# Autodesk Inventor assembly: MovingArm
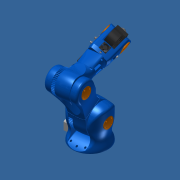
[picture p0: Inventor's stored thumbnail of the model, 180x180]
Saved by Autodesk Inventor 2014 SP2 (Build 180246200, 246)
## iProperties
Created: 2014-12-13
Part Number: MovingArm
Document SubType Name: Assembly
Designer: 4ndreas
Author: 4ndreas
## Documents named in this file (22)
- C:\Users\4ndreas\Documents\Inventor\RobotARm\MovingArm.iam
- C:\Users\4ndreas\Documents\Inventor\RobotARm\Nema17.ipt
- C:\Users\4ndreas\Documents\Inventor\Content Center Files\R2014\de-DE\DIN BEARING(1)\DIN 625 SKF - SKF 608.ipt
- C:\Users\4ndreas\Documents\Inventor\Content Center Files\R2014\de-DE\DIN 931-1\DIN 931-1 - M8 x 60.ipt
- C:\Users\4ndreas\Documents\Inventor\RobotARm\ArmSegment_klein_Gear.ipt
- C:\Users\4ndreas\Documents\Inventor\RobotARm\ArmSegment_klein.ipt
- C:\Users\4ndreas\Documents\Inventor\RobotARm\Nema17 Geared.ipt
- C:\Users\4ndreas\Documents\Inventor\RobotARm\Abdeckung.ipt
- C:\Users\4ndreas\Documents\Inventor\RobotARm\print\ArmPrint_A.ipt
- C:\Users\4ndreas\Documents\Inventor\RobotARm\print\ArmPrint_B_gear.ipt
- C:\Users\4ndreas\Documents\Inventor\RobotARm\print\ArmPrint_C_head.ipt
- C:\Users\4ndreas\Documents\Inventor\RobotARm\Stirnzahnrad_A_print.ipt
- C:\Users\4ndreas\Documents\Inventor\RobotARm\Stirnzahnrad_B_print.ipt
- C:\Users\4ndreas\Documents\Inventor\RobotARm\print\basis_print.ipt
- C:\Users\4ndreas\Documents\Inventor\RobotARm\foreArm.iam
- C:\Users\4ndreas\Documents\Inventor\Content Center Files\R2014\Leufter_30mm.ipt
- C:\Users\4ndreas\Documents\Inventor\RobotARm\MovingArm\AIP\FEA\b9sg0glls.fins
- C:\Users\4ndreas\Documents\Inventor\RobotARm\MovingArm\AIP\FEA\b9sg0glls.fsat
- C:\Users\4ndreas\Documents\Inventor\RobotARm\MovingArm\AIP\FEA\b9sg0glls.ftes
- C:\Users\4ndreas\Documents\Inventor\RobotARm\MovingArm\AIP\FEA\b9sg0glls.fwiz
- C:\Users\4ndreas\Documents\Inventor\RobotARm\MovingArm\AIP\FEA\b9sg0glxc.fmsh
- C:\Users\4ndreas\Documents\Inventor\RobotARm\MovingArm\AIP\FEA\b9sg0glxd.fres
## Components (23 placed, 15 different names)
1. basis_print:1 — Passend:1, Passend:2, Passend:4, Passend:6, Passend:7, Passend:8, Passend:9, Passend:10, Passend:11, Passend:12, Passend:13, Passend:14, Passend:43, Passend:44, Passend:45, Passend:46, Passend:47, Passend:48, Passend:50, Passend:69
2. Nema17:1 — Passend:5, Passend:6, Passend:67, Passend:69
3. DIN 625 SKF 608:1 — Passend:8, Passend:13
4. DIN 625 SKF 608:2 — Passend:7, Passend:14, Passend:15, Passend:18
5. DIN 625 SKF 608:3 — Passend:10, Passend:12, Passend:16, Passend:17
6. DIN 625 SKF 608:4 — Passend:9, Passend:11
7. DIN 931-1 - ersetzt durch DIN EN 24014 M8 x 60:1 — Passend:16, Passend:17, Passend:49
8. DIN 931-1 - ersetzt durch DIN EN 24014 M8 x 60:2 — Passend:15, Passend:18, Passend:51
9. Nema17:2 — Passend:56, Passend:59, Passend:60, Passend:68
10. ArmSegment_klein_Gear:1 — Passend:27, Passend:28, Passend:29, Passend:30, Passend:31, Passend:32, Passend:57, Passend:58, Fluchtend:3, Passend:72, Passend:73, Passend:76
11. ArmSegment_klein:1 — Passend:30, Passend:31, Passend:32, Passend:71
12. Nema17 Geared:1 — Passend:27, Passend:28, Passend:29, Passend:70
13. Abdeckung:1 — Passend:61, Passend:65, Passend:66
14. Abdeckung:2 — Passend:44, Passend:45, Passend:46
15. Abdeckung:3 — Passend:62, Passend:63, Passend:64
16. Abdeckung:4 — Passend:43, Passend:47, Passend:48
17. ArmPrint_A:1 — Passend:49, Passend:50, Passend:52, Fluchtend:1, Passend:55, Passend:62
18. ArmPrint_B_gear:1 — Passend:51, Passend:52, Fluchtend:1, Passend:53, Passend:54, Fluchtend:2
19. ArmPrint_C_head:1 — Passend:53, Passend:54, Passend:55, Passend:56, Passend:57, Passend:58, Passend:59, Passend:60, Passend:61, Passend:63, Passend:64, Passend:65, Passend:66
20. Stirnzahnrad_A_print:1 — Passend:67, Fluchtend:2
21. Stirnzahnrad_B_print:1 — Passend:68, Fluchtend:3
22. foreArm:1 [sub-assembly] — Passend:70, Passend:71
23. Leufter_30mm:1 — Passend:72, Passend:73, Passend:74, Passend:75
## Relationships (60: Mate 57, Flush 3)
- Passend:1 [Mate]: basis_print:1
- Passend:2 [Mate]: basis_print:1
- Passend:4 [Mate]: basis_print:1
- Passend:5 [Mate]: Nema17:1
- Passend:6 [Mate]: basis_print:1 ↔ Nema17:1
- Passend:7 [Mate]: basis_print:1 ↔ DIN 625 SKF 608:2
- Passend:8 [Mate]: basis_print:1 ↔ DIN 625 SKF 608:1
- Passend:9 [Mate]: basis_print:1 ↔ DIN 625 SKF 608:4
- Passend:10 [Mate]: basis_print:1 ↔ DIN 625 SKF 608:3
- Passend:11 [Mate]: basis_print:1 ↔ DIN 625 SKF 608:4
- Passend:12 [Mate]: basis_print:1 ↔ DIN 625 SKF 608:3
- Passend:13 [Mate]: basis_print:1 ↔ DIN 625 SKF 608:1
- Passend:14 [Mate]: basis_print:1 ↔ DIN 625 SKF 608:2
- Passend:15 [Mate]: DIN 625 SKF 608:2 ↔ DIN 931-1 - ersetzt durch DIN EN 24014 M8 x 60:2
- Passend:16 [Mate]: DIN 625 SKF 608:3 ↔ DIN 931-1 - ersetzt durch DIN EN 24014 M8 x 60:1
- Passend:17 [Mate]: DIN 625 SKF 608:3 ↔ DIN 931-1 - ersetzt durch DIN EN 24014 M8 x 60:1
- Passend:18 [Mate]: DIN 625 SKF 608:2 ↔ DIN 931-1 - ersetzt durch DIN EN 24014 M8 x 60:2
- Passend:27 [Mate]: ArmSegment_klein_Gear:1 ↔ Nema17 Geared:1
- Passend:28 [Mate]: ArmSegment_klein_Gear:1 ↔ Nema17 Geared:1
- Passend:29 [Mate]: ArmSegment_klein_Gear:1 ↔ Nema17 Geared:1
- Passend:30 [Mate]: ArmSegment_klein_Gear:1 ↔ ArmSegment_klein:1
- Passend:31 [Mate]: ArmSegment_klein_Gear:1 ↔ ArmSegment_klein:1
- Passend:32 [Mate]: ArmSegment_klein_Gear:1 ↔ ArmSegment_klein:1
- Passend:43 [Mate]: basis_print:1 ↔ Abdeckung:4
- Passend:44 [Mate]: basis_print:1 ↔ Abdeckung:2
- Passend:45 [Mate]: basis_print:1 ↔ Abdeckung:2
- Passend:46 [Mate]: basis_print:1 ↔ Abdeckung:2
- Passend:47 [Mate]: basis_print:1 ↔ Abdeckung:4
- Passend:48 [Mate]: basis_print:1 ↔ Abdeckung:4
- Passend:49 [Mate]: DIN 931-1 - ersetzt durch DIN EN 24014 M8 x 60:1 ↔ ArmPrint_A:1
- Passend:50 [Mate] (3 mm): basis_print:1 ↔ ArmPrint_A:1
- Passend:51 [Mate]: DIN 931-1 - ersetzt durch DIN EN 24014 M8 x 60:2 ↔ ArmPrint_B_gear:1
- Passend:52 [Mate]: ArmPrint_A:1 ↔ ArmPrint_B_gear:1
- Fluchtend:1 [Flush]: ArmPrint_A:1 ↔ ArmPrint_B_gear:1
- Passend:53 [Mate]: ArmPrint_B_gear:1 ↔ ArmPrint_C_head:1
- Passend:54 [Mate]: ArmPrint_B_gear:1 ↔ ArmPrint_C_head:1
- Passend:55 [Mate]: ArmPrint_A:1 ↔ ArmPrint_C_head:1
- Passend:56 [Mate]: Nema17:2 ↔ ArmPrint_C_head:1
- Passend:57 [Mate]: ArmSegment_klein_Gear:1 ↔ ArmPrint_C_head:1
- Passend:58 [Mate] (2 mm): ArmSegment_klein_Gear:1 ↔ ArmPrint_C_head:1
- Passend:59 [Mate]: Nema17:2 ↔ ArmPrint_C_head:1
- Passend:60 [Mate]: Nema17:2 ↔ ArmPrint_C_head:1
- Passend:61 [Mate]: Abdeckung:1 ↔ ArmPrint_C_head:1
- Passend:62 [Mate]: Abdeckung:3 ↔ ArmPrint_A:1
- Passend:63 [Mate]: Abdeckung:3 ↔ ArmPrint_C_head:1
- Passend:64 [Mate]: Abdeckung:3 ↔ ArmPrint_C_head:1
- Passend:65 [Mate]: Abdeckung:1 ↔ ArmPrint_C_head:1
- Passend:66 [Mate]: Abdeckung:1 ↔ ArmPrint_C_head:1
- Passend:67 [Mate]: Nema17:1 ↔ Stirnzahnrad_A_print:1
- Fluchtend:2 [Flush] (-1 mm): ArmPrint_B_gear:1 ↔ Stirnzahnrad_A_print:1
- Passend:68 [Mate]: Nema17:2 ↔ Stirnzahnrad_B_print:1
- Fluchtend:3 [Flush]: ArmSegment_klein_Gear:1 ↔ Stirnzahnrad_B_print:1
- Passend:69 [Mate]: basis_print:1 ↔ Nema17:1
- Passend:70 [Mate]: Nema17 Geared:1 ↔ foreArm:1
- Passend:71 [Mate] (2 mm): ArmSegment_klein:1 ↔ foreArm:1
- Passend:72 [Mate]: ArmSegment_klein_Gear:1 ↔ Leufter_30mm:1
- Passend:73 [Mate]: ArmSegment_klein_Gear:1 ↔ Leufter_30mm:1
- Passend:74 [Mate]: Leufter_30mm:1
- Passend:75 [Mate]: Leufter_30mm:1
- Passend:76 [Mate]: ArmSegment_klein_Gear:1
